# Autodesk Inventor assembly: Assembly1
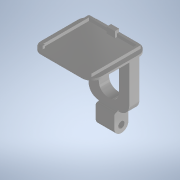
[picture p0: Inventor's stored thumbnail of the model, 180x180]
Saved by Autodesk Inventor 2022.1 (Build 261234020, 234B)
## iProperties
Created: 2021-10-31
Part Number: Assembly1
Document SubType Name: Assembly
Designer: 46734
Author: 46734
## Documents named in this file (3)
- G:\Min enhet\GA\3d print\Assembly1.iam
- C:\Users\46734\Downloads\GAkameraback v1.ipt
- C:\Users\46734\Downloads\GAkamerakropp v1.ipt
## Components (2 placed, 2 different names)
1. GAkameraback v1:1 — Mate:1, Flush:1, Flush:2
2. GAkamerakropp v1:1 — Mate:1, Flush:1, Flush:2
## Relationships (3: Flush 2, Mate 1)
- Mate:1: GAkameraback v1:1 ↔ GAkamerakropp v1:1
- Flush:1 (-1.5 mm): GAkameraback v1:1 ↔ GAkamerakropp v1:1
- Flush:2 (2.4 mm): GAkameraback v1:1 ↔ GAkamerakropp v1:1
